# Autodesk Inventor assembly: 150G_FLIPPER_ASSY_001
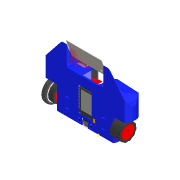
[picture p0: Inventor's stored thumbnail of the model, 180x180]
Saved by Autodesk Inventor 2020 (Build 240168000, 168)
## iProperties
Created: 2018-10-31
Part Number: 150G_FLIPPER_ASSY_001
Description: STEP AP214
Document SubType Name: Assembly
Designer: darioneuenschwander
Sending System: SolidWorks 2018
Preprocessor: SwSTEP 2.0
Title: 150G_FLIPPER_ASSY_001.STEP
Revision Number: ANY
## Documents named in this file (22)
- \\Mac\Home\Desktop\CAD\Antweight\Flipper\150G_FLIPPER_ASSY_001.iam
- \\Mac\Home\Desktop\CAD\Antweight\Flipper\150_flipper_base_001.ipt
- \\Mac\Home\Desktop\CAD\Antweight\Flipper\Pololu - 1_250 Micro gear motor.ipt
- \\Mac\Home\Desktop\CAD\Antweight\Flipper\24MMWHEEL.ipt
- \\Mac\Home\Desktop\CAD\Antweight\Flipper\ServoTGY-306GV2.2_Dfaut.ipt
- \\Mac\Home\Desktop\CAD\Antweight\Flipper\Turnigy 300mah 2s.ipt
- \\Mac\Home\Desktop\CAD\Antweight\Flipper\Servo Arm HXT900 Micro.ipt
- \\Mac\Home\Desktop\CAD\Antweight\Flipper\flipper_arm_002.ipt
- \\Mac\Home\Desktop\CAD\Antweight\Flipper\flipper_lever.ipt
- \\Mac\Home\Desktop\CAD\Antweight\Flipper\flipper_wedge.ipt
- \\Mac\Home\Desktop\CAD\Antweight\Flipper\flipper_wedge_18mm.ipt
- \\Mac\Home\Desktop\CAD\Antweight\Flipper\Budget DESC.ipt
- \\Mac\Home\Desktop\CAD\Antweight\Flipper\90380A106_PHILLIPS THREAD-FORMING SCREW FOR PLASTIC_90380A106.ipt
- \\Mac\Home\Desktop\CAD\Antweight\Flipper\top_plate_LEFT.ipt
- \\Mac\Home\Desktop\CAD\Antweight\Flipper\top_plate_RIGHT.ipt
- \\Mac\Home\Desktop\CAD\Antweight\Flipper\24mmlegohub.ipt
- \\Mac\Home\Desktop\CAD\Antweight\Flipper\50mmrod.ipt
- \\Mac\Home\Desktop\CAD\Antweight\Flipper\top cover.ipt
- \\Mac\Home\Desktop\CAD\Antweight\Flipper\spacer.ipt
- \\Mac\Home\Desktop\CAD\Antweight\Flipper\spacer_wide.ipt
- \\Mac\Home\Desktop\CAD\Antweight\ttgo-t-display.iam
- \\Mac\Home\Desktop\CAD\Antweight\Mäher\Pololu-Wheel-32x7mm___ _________.iam
## Components (40 placed, 40 different names)
1. 150_flipper_base_001_1 — Fluchtend:1, Fluchtend:2, Passend:6, Passend:7, Passend:8, Fluchtend:3, Passend:11
2. Pololu - 1_250 Micro gear motor_2 — Passend:6, Passend:7
3. Pololu - 1_250 Micro gear motor_3 — Passend:8
4. 24MMWHEEL_4
5. 24MMWHEEL_5
6. ServoTGY-306GV2.2_Dfaut_6 — Fluchtend:2, Passend:5, Fluchtend:3, Passend:11
7. Turnigy 300mah 2s_7
8. Servo Arm HXT900 Micro_8 — Passend:5
9. flipper_arm_002_9
10. flipper_arm_002_10
11. flipper_lever_11
12. flipper_wedge_12
13. flipper_wedge_18mm_13
14. Budget DESC_14
15. 90380A106_PHILLIPS THREAD-FORMING SCREW FOR PLASTIC_90380A106_15
16. 90380A106_PHILLIPS THREAD-FORMING SCREW FOR PLASTIC_90380A106_16
17. 90380A106_PHILLIPS THREAD-FORMING SCREW FOR PLASTIC_90380A106_17
18. 90380A106_PHILLIPS THREAD-FORMING SCREW FOR PLASTIC_90380A106_18
19. 90380A106_PHILLIPS THREAD-FORMING SCREW FOR PLASTIC_90380A106_19
20. 90380A106_PHILLIPS THREAD-FORMING SCREW FOR PLASTIC_90380A106_20
21. 90380A106_PHILLIPS THREAD-FORMING SCREW FOR PLASTIC_90380A106_21
22. 90380A106_PHILLIPS THREAD-FORMING SCREW FOR PLASTIC_90380A106_22
23. top_plate_LEFT_23
24. top_plate_RIGHT_24
25. 24mmlegohub_25 — Passend:10
26. 24mmlegohub_26
27. 90380A106_PHILLIPS THREAD-FORMING SCREW FOR PLASTIC_90380A106_27
28. 90380A106_PHILLIPS THREAD-FORMING SCREW FOR PLASTIC_90380A106_28
29. 90380A106_PHILLIPS THREAD-FORMING SCREW FOR PLASTIC_90380A106_29
30. 90380A106_PHILLIPS THREAD-FORMING SCREW FOR PLASTIC_90380A106_30
31. 50mmrod_31
32. top cover_32
33. 90380A106_PHILLIPS THREAD-FORMING SCREW FOR PLASTIC_90380A106_33
34. 90380A106_PHILLIPS THREAD-FORMING SCREW FOR PLASTIC_90380A106_34
35. 90380A106_PHILLIPS THREAD-FORMING SCREW FOR PLASTIC_90380A106_35
36. 90380A106_PHILLIPS THREAD-FORMING SCREW FOR PLASTIC_90380A106_36
37. spacer_37
38. spacer_wide_38
39. ttgo-t-display:1 [sub-assembly] — Fluchtend:1
40. Pololu-Wheel-32x7mm___ _________:1 [sub-assembly] — Passend:10
## Relationships (9: Mate 6, Flush 3)
- Fluchtend:1 [Flush] (2 mm): 150_flipper_base_001_1 ↔ ttgo-t-display:1
- Fluchtend:2 [Flush] (3 mm): 150_flipper_base_001_1 ↔ ServoTGY-306GV2.2_Dfaut_6
- Passend:5 [Mate]: ServoTGY-306GV2.2_Dfaut_6 ↔ Servo Arm HXT900 Micro_8
- Passend:6 [Mate]: 150_flipper_base_001_1 ↔ Pololu - 1_250 Micro gear motor_2
- Passend:7 [Mate]: 150_flipper_base_001_1 ↔ Pololu - 1_250 Micro gear motor_2
- Passend:8 [Mate]: 150_flipper_base_001_1 ↔ Pololu - 1_250 Micro gear motor_3
- Passend:10 [Mate]: 24mmlegohub_25 ↔ Pololu-Wheel-32x7mm___ _________:1
- Fluchtend:3 [Flush]: 150_flipper_base_001_1 ↔ ServoTGY-306GV2.2_Dfaut_6
- Passend:11 [Mate] (1.5 mm): 150_flipper_base_001_1 ↔ ServoTGY-306GV2.2_Dfaut_6
